# Autodesk Inventor assembly: S8x1
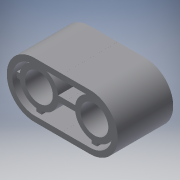
[picture p0: Inventor's stored thumbnail of the model, 180x180]
Saved by Autodesk Inventor 2019 (Build 230136000, 136)
## iProperties
Created: 2019-01-31
Part Number: S8x1
Document SubType Name: Assembly
Designer: Varga Daniel
Author: Varga Daniel
## Documents named in this file (2)
- C:\!_Dani\!_cloud\OneDrive\!_munka\Revolution\RevvyDemoKit\Structural parts\Straight Beams\S2x1.iam
- C:\!_Dani\!_cloud\OneDrive\!_munka\Revolution\RevvyDemoKit\Structural parts\Straight Beams\straight_beam_end_part_single.ipt
## Components (2 placed, 1 different names)
1. straight_beam_end_part_single:1 — Flush:1, Flush:2, Mate:1
2. straight_beam_end_part_single:2 — Flush:1, Flush:2, Mate:1
## Relationships (3: Flush 2, Mate 1)
- Flush:1: straight_beam_end_part_single:1 ↔ straight_beam_end_part_single:2
- Flush:2: straight_beam_end_part_single:1 ↔ straight_beam_end_part_single:2
- Mate:1: straight_beam_end_part_single:1 ↔ straight_beam_end_part_single:2
